# Autodesk Inventor assembly: outer box
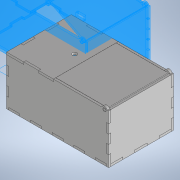
[picture p0: Inventor's stored thumbnail of the model, 180x180]
Saved by Autodesk Inventor 2020 (Build 240168000, 168)
## iProperties
Created: 2022-02-14
Part Number: outer box
Document SubType Name: Assembly
Designer: rwte
Author: rwte
## Documents named in this file (8)
- C:\Users\carl\Documents\GitHub\CAD\final project\ipt files\outer box.iam
- C:\Users\carl\Documents\GitHub\CAD\final project\ipt files\bottom.ipt
- C:\Users\carl\Documents\GitHub\CAD\final project\ipt files\Wall 1.ipt
- C:\Users\carl\Documents\GitHub\CAD\final project\ipt files\back.ipt
- C:\Users\carl\Documents\GitHub\CAD\final project\ipt files\Front.ipt
- C:\Users\carl\Documents\GitHub\CAD\final project\ipt files\top switch.ipt
- C:\Users\carl\Documents\GitHub\CAD\final project\ipt files\top lid.ipt
- C:\Users\carl\Documents\GitHub\CAD\final project\ipt files\wall 2.ipt
## Components (7 placed, 7 different names)
1. bottom:1 — Mate:1, Mate:2, Mate:3, Mate:6
2. Wall 1:1 — Mate:1, Mate:2, Mate:3, Mate:4, Mate:5, Mate:7, Mate:8, Mate:9
3. back:1 — Mate:6, Mate:7
4. Front:1 — Mate:4, Mate:5, Mate:13, Mate:14
5. top switch:1 — Mate:8, Mate:9
6. top lid:1 — Rotational:1
7. wall 2:1 — Mate:13, Mate:14, Rotational:1
## Relationships (12: Mate 11, RevoluteJoint 1)
- Mate:1: bottom:1 ↔ Wall 1:1
- Mate:2: bottom:1 ↔ Wall 1:1
- Mate:3: bottom:1 ↔ Wall 1:1
- Mate:4: Wall 1:1 ↔ Front:1
- Mate:5: Wall 1:1 ↔ Front:1
- Mate:6: bottom:1 ↔ back:1
- Mate:7: Wall 1:1 ↔ back:1
- Mate:8: Wall 1:1 ↔ top switch:1
- Mate:9: Wall 1:1 ↔ top switch:1
- Mate:13: Front:1 ↔ wall 2:1
- Mate:14: Front:1 ↔ wall 2:1
- Rotational:1 [RevoluteJoint]: top lid:1 ↔ wall 2:1
